# Autodesk Inventor assembly: Stepper with bracket
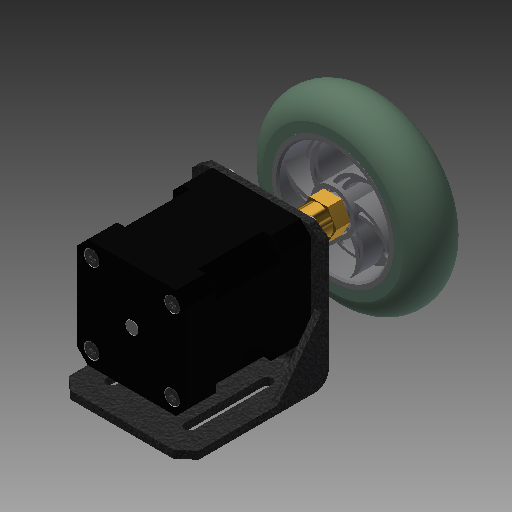
[picture p0: Inventor's stored thumbnail of the model, 512x512]
Saved by Autodesk Inventor 2018 (Build 220112000, 112)
## iProperties
Created: 2018-05-02
Part Number: Stepper with bracket
Document SubType Name: Assembly
Designer: Ajith Thomas
Author: Ajith Thomas
## Documents named in this file (4)
- C:\Users\Ajith Thomas\Dropbox\Gas_Sensing_Robot\FumeBot-Design\Stepper with bracket.iam
- C:\Users\Ajith Thomas\Dropbox\Gas_Sensing_Robot\FumeBot-Design\Stepper Motor\Stepper Bracket.ipt
- C:\Users\Ajith Thomas\Dropbox\Gas_Sensing_Robot\FumeBot-Design\Stepper with wheel.iam
- C:\Users\Ajith Thomas\Documents\Inventor\Content Center Files\R2018\en-US\ISO 4762(1)\DIN EN ISO 4762 - M3 x 6.ipt
## Components (6 placed, 3 different names)
1. Stepper Bracket:1 — Mate:1, Mate:2, Mate:3, Insert:1, Insert:2, Insert:3, Insert:4
2. Stepper with wheel:1 [sub-assembly] — Mate:1, Mate:2, Mate:3
3. DIN EN ISO 4762 M3 x 6:1 — Insert:1
4. DIN EN ISO 4762 M3 x 6:2 — Insert:2
5. DIN EN ISO 4762 M3 x 6:3 — Insert:3
6. DIN EN ISO 4762 M3 x 6:4 — Insert:4
## Relationships (7: Insert 4, Mate 3)
- Mate:1: Stepper Bracket:1 ↔ Stepper with wheel:1
- Mate:2: Stepper Bracket:1 ↔ Stepper with wheel:1
- Mate:3: Stepper Bracket:1 ↔ Stepper with wheel:1
- Insert:1: Stepper Bracket:1 ↔ DIN EN ISO 4762 M3 x 6:1
- Insert:2: Stepper Bracket:1 ↔ DIN EN ISO 4762 M3 x 6:2
- Insert:3: Stepper Bracket:1 ↔ DIN EN ISO 4762 M3 x 6:3
- Insert:4: Stepper Bracket:1 ↔ DIN EN ISO 4762 M3 x 6:4
